# Autodesk Inventor assembly: Air2D
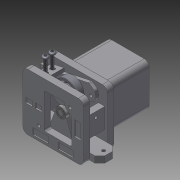
[picture p0: Inventor's stored thumbnail of the model, 180x180]
Saved by Autodesk Inventor 2014 (Build 180170000, 170)
## iProperties
Created: 2014-09-30
Part Number: Air2D
Document SubType Name: Assembly
Designer: ThatOtherGuy
Author: ThatOtherGuy
## Documents named in this file (16)
- U:\Hobbies\Inventor\KosselCNC1515\Extruder\Air2D.iam
- U:\Hobbies\Inventor\KosselCNC1515\Extruder\Air2D_Front_Feed.ipt
- U:\Hobbies\Inventor\KosselCNC1515\Extruder\Air2D_Side_Motor.ipt
- U:\Hobbies\Inventor\KosselCNC1515\Extruder\Air2D_Back_Bowden.ipt
- U:\Hobbies\Inventor\KosselCNC1515\NEMA17.ipt
- U:\Hobbies\Inventor\KosselCNC1515\Extruder\Air2D_Hinge_Sideplate.ipt
- U:\Hobbies\Inventor\Content Center Files\R2014\en-US\DIN 625 SKF(4)\DIN 625 SKF - SKF 608-2Z.ipt
- U:\Hobbies\Inventor\KosselCNC1515\Extruder\Air2D_Hinge_Top.ipt
- U:\Hobbies\Inventor\Content Center Files\R2014\en-US\ANSI B18.3.4M(1)\ANSI B18.3.4M - M3 x 0.5 x 45(2).ipt
- U:\Hobbies\Inventor\Content Center Files\R2014\en-US\ISO 10511\ISO 10511 - M3.ipt
- U:\Hobbies\Inventor\KosselCNC1515\Extruder\Air2D_Bottom.ipt
- U:\Hobbies\Inventor\KosselCNC1515\Extruder\Air2D_Side_Face.ipt
- U:\Hobbies\Inventor\KosselCNC1515\Extruder\MK8_Drive_Gear.ipt
- U:\Hobbies\Inventor\KosselCNC1515\Bearing 2ZZ (Metric)\Bearing 5x10x4-2Z.ipt
- C:\Users\ThatOtherGuy\Documents\Inventor\KosselCNC1515\Bearing 2ZZ (Metric).ipt
- U:\Hobbies\Inventor\KosselCNC1515\Extruder\Air2D_Shaft_Brace.ipt
## Components (18 placed, 14 different names)
1. Air2D_Side_Motor:1 — Mate:1, Mate:2, Mate:3, Mate:4, Mate:6, Mate:7, Mate:8, Mate:9, Mate:10, Mate:19, Mate:20, Mate:25, Mate:26, Mate:27, Mate:32, Angle:2
2. Air2D_Front_Feed:1 — Mate:1, Mate:2, Mate:3, Flush:1
3. Air2D_Back_Bowden:1 — Flush:1, Mate:4, Mate:19, Flush:5, Flush:6, Tangent:5
4. NEMA17:1 — Mate:6, Mate:7, Mate:8, Mate:35, Mate:36, Mate:43
5. Air2D_Hinge_Sideplate:1 — Mate:9, Mate:10, Mate:11, Mate:12, Mate:17, Mate:18
6. DIN 625 SKF- with two Z shields SKF 608-2Z:1 — Mate:11, Mate:12, Tangent:8
7. Air2D_Hinge_Sideplate:2 — Mate:17, Mate:18, Mate:39, Mate:40, Flush:9
8. Air2D_Back_Bowden:2 — Flush:5, Flush:6, Mate:20, Tangent:2, Flush:7, Mate:37, Mate:38
9. Broached Hexagon Socket Button Head Cap Screw - Metric M3 x 0.5 x 45:1 — Tangent:2, Flush:7, Mate:23, Flush:8, Tangent:9
10. Broached Hexagon Socket Button Head Cap Screw - Metric M3 x 0.5 x 45:2 — Tangent:5, Flush:8, Tangent:10, Mate:42
11. DIN EN ISO 10511 M3:1 — Mate:23, Mate:37, Angle:1, Angle:2
12. Air2D_Bottom:1 — Mate:25, Mate:26, Mate:27, Mate:34, Mate:41, Mate:45
13. DIN EN ISO 10511 M3:2 — Mate:38, Angle:1
14. Air2D_Side_Face:1 — Mate:32, Mate:34, Mate:39, Mate:41, Mate:44, Mate:46
15. MK8_Drive_Gear:1 — Mate:35, Mate:36, Tangent:8
16. Air2D_Hinge_Top:1 — Mate:40, Flush:9, Tangent:9, Tangent:10, Mate:42
17. Bearing 5x10x4-2Z:1 — Mate:43, Mate:44, Tangent:11
18. Air2D_Shaft_Brace:1 — Mate:45, Mate:46, Tangent:11
## Relationships (48: Mate 34, Flush 6, Tangent 6, Angle 2)
- Mate:1: Air2D_Side_Motor:1 ↔ Air2D_Front_Feed:1
- Mate:2: Air2D_Side_Motor:1 ↔ Air2D_Front_Feed:1
- Mate:3: Air2D_Side_Motor:1 ↔ Air2D_Front_Feed:1
- Flush:1: Air2D_Front_Feed:1 ↔ Air2D_Back_Bowden:1
- Mate:4: Air2D_Side_Motor:1 ↔ Air2D_Back_Bowden:1
- Mate:6: Air2D_Side_Motor:1 ↔ NEMA17:1
- Mate:7: Air2D_Side_Motor:1 ↔ NEMA17:1
- Mate:8: Air2D_Side_Motor:1 ↔ NEMA17:1
- Mate:9: Air2D_Side_Motor:1 ↔ Air2D_Hinge_Sideplate:1
- Mate:10: Air2D_Side_Motor:1 ↔ Air2D_Hinge_Sideplate:1
- Mate:11: Air2D_Hinge_Sideplate:1 ↔ DIN 625 SKF- with two Z shields SKF 608-2Z:1
- Mate:12 (2 mm): Air2D_Hinge_Sideplate:1 ↔ DIN 625 SKF- with two Z shields SKF 608-2Z:1
- Mate:17: Air2D_Hinge_Sideplate:1 ↔ Air2D_Hinge_Sideplate:2
- Mate:18: Air2D_Hinge_Sideplate:1 ↔ Air2D_Hinge_Sideplate:2
- Mate:19: Air2D_Side_Motor:1 ↔ Air2D_Back_Bowden:1
- Flush:5: Air2D_Back_Bowden:1 ↔ Air2D_Back_Bowden:2
- Flush:6: Air2D_Back_Bowden:1 ↔ Air2D_Back_Bowden:2
- Mate:20: Air2D_Side_Motor:1 ↔ Air2D_Back_Bowden:2
- Tangent:2: Air2D_Back_Bowden:2 ↔ Broached Hexagon Socket Button Head Cap Screw - Metric M3 x 0.5 x 45:1
- Flush:7 (-5 mm): Air2D_Back_Bowden:2 ↔ Broached Hexagon Socket Button Head Cap Screw - Metric M3 x 0.5 x 45:1
- Mate:23: Broached Hexagon Socket Button Head Cap Screw - Metric M3 x 0.5 x 45:1 ↔ DIN EN ISO 10511 M3:1
- Mate:25: Air2D_Side_Motor:1 ↔ Air2D_Bottom:1
- Mate:26: Air2D_Side_Motor:1 ↔ Air2D_Bottom:1
- Mate:27: Air2D_Side_Motor:1 ↔ Air2D_Bottom:1
- [Mate]: Broached Hexagon Socket Button Head Cap Screw - Metric M3 x 0.5 x 45:2 ↔ DIN EN ISO 10511 M3:2
- Tangent:5: Air2D_Back_Bowden:1 ↔ Broached Hexagon Socket Button Head Cap Screw - Metric M3 x 0.5 x 45:2
- Flush:8: Broached Hexagon Socket Button Head Cap Screw - Metric M3 x 0.5 x 45:1 ↔ Broached Hexagon Socket Button Head Cap Screw - Metric M3 x 0.5 x 45:2
- Mate:32: Air2D_Side_Motor:1 ↔ Air2D_Side_Face:1
- Mate:34: Air2D_Bottom:1 ↔ Air2D_Side_Face:1
- Mate:35: NEMA17:1 ↔ MK8_Drive_Gear:1
- Mate:36 (5.5 mm): NEMA17:1 ↔ MK8_Drive_Gear:1
- Mate:37: Air2D_Back_Bowden:2 ↔ DIN EN ISO 10511 M3:1
- Mate:38: Air2D_Back_Bowden:2 ↔ DIN EN ISO 10511 M3:2
- Mate:39: Air2D_Hinge_Sideplate:2 ↔ Air2D_Side_Face:1
- Tangent:8: DIN 625 SKF- with two Z shields SKF 608-2Z:1 ↔ MK8_Drive_Gear:1
- Mate:40: Air2D_Hinge_Sideplate:2 ↔ Air2D_Hinge_Top:1
- Flush:9: Air2D_Hinge_Sideplate:2 ↔ Air2D_Hinge_Top:1
- Tangent:9 (0.1 mm): Broached Hexagon Socket Button Head Cap Screw - Metric M3 x 0.5 x 45:1 ↔ Air2D_Hinge_Top:1
- Tangent:10 (0.1 mm): Broached Hexagon Socket Button Head Cap Screw - Metric M3 x 0.5 x 45:2 ↔ Air2D_Hinge_Top:1
- Angle:1 (0 deg): DIN EN ISO 10511 M3:1 ↔ DIN EN ISO 10511 M3:2
- Angle:2 (0 deg): Air2D_Side_Motor:1 ↔ DIN EN ISO 10511 M3:1
- Mate:41: Air2D_Bottom:1 ↔ Air2D_Side_Face:1
- Mate:42 (1 mm): Broached Hexagon Socket Button Head Cap Screw - Metric M3 x 0.5 x 45:2 ↔ Air2D_Hinge_Top:1
- Mate:43: NEMA17:1 ↔ Bearing 5x10x4-2Z:1
- Mate:44: Air2D_Side_Face:1 ↔ Bearing 5x10x4-2Z:1
- Mate:45: Air2D_Bottom:1 ↔ Air2D_Shaft_Brace:1
- Mate:46: Air2D_Side_Face:1 ↔ Air2D_Shaft_Brace:1
- Tangent:11: Bearing 5x10x4-2Z:1 ↔ Air2D_Shaft_Brace:1
## Named parameters: d40_d34 = 0 mm
